# Autodesk Inventor assembly: printer
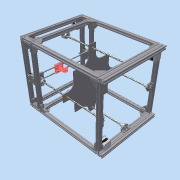
[picture p0: Inventor's stored thumbnail of the model, 180x180]
Saved by Autodesk Inventor 2015 (Build 190159000, 159)
## iProperties
Created: 2016-06-24
Part Number: printer
Document SubType Name: Assembly
Designer: Dustin
Author: Dustin
## Documents named in this file (25)
- E:\Documents\3D Printer\Parts\New Printer\printer.iam
- E:\Documents\3D Printer\Parts\New Printer\20x20x9in.ipt
- E:\Documents\3D Printer\Parts\New Printer\20x20x27cm.ipt
- E:\Documents\3D Printer\Parts\New Printer\heated bed.ipt
- E:\Documents\3D Printer\Parts\New Printer\NEMA17.ipt
- E:\Documents\3D Printer\Parts\New Printer\.375 - 8 (4 start) acme thread.ipt
- E:\Documents\3D Printer\Parts\New Printer\leadscrew corners.ipt
- E:\Documents\3D Printer\Parts\New Printer\bed plate.ipt
- E:\Documents\3D Printer\Parts\New Printer\Imported Components\GT2_20teeth_pulley\GT2_20teeth_pulley.ipt
- E:\Documents\3D Printer\Parts\New Printer\6mm_rod_265.ipt
- E:\Documents\3D Printer\Parts\New Printer\motor mount.ipt
- E:\Documents\3D Printer\Parts\New Printer\20x20x5cm.ipt
- E:\Documents\3D Printer\Parts\New Printer\extruder.iam
- E:\Documents\3D Printer\Parts\New Printer\X smooth mount.ipt
- E:\Documents\3D Printer\Parts\New Printer\m3x20.ipt
- E:\Documents\3D Printer\Parts\New Printer\Corner mount.ipt
- E:\Documents\3D Printer\Parts\New Printer\m4 bearing assembly.iam
- E:\Documents\3D Printer\Parts\New Printer\m4 bearing assembly 30mm.iam
- E:\Documents\3D Printer\Parts\New Printer\KFL08.iam
- E:\Documents\3D Printer\Parts\New Printer\vwheel.iam
- E:\Documents\3D Printer\Parts\New Printer\m5x16m.ipt
- E:\Documents\3D Printer\Parts\New Printer\m8 nut.ipt
- E:\Documents\3D Printer\Parts\New Printer\corners.ipt
- E:\Documents\3D Printer\Parts\New Printer\Corner mount_MIR.ipt
- E:\Documents\3D Printer\Parts\New Printer\corner bracket.ipt
## Components (123 placed, 25 different names)
1. 20x20x9in:2 — Mate:4, Flush:8, Flush:9, Mate:6, Mate:39, Flush:53, Flush:64, Mate:66, Mate:113, Flush:122, Angle:30
2. 20x20x9in:3 — Mate:5, Flush:10, Flush:11, Flush:12, Flush:13, Mate:48, Flush:51, Flush:65, Mate:67, Mate:109, Flush:120
3. 20x20x27cm:3 — Mate:4, Flush:8, Flush:9, Mate:5, Flush:10, Flush:11, Mate:11, Mate:12, Flush:24, Flush:25, Flush:26, Flush:27, Mate:60, Flush:60, Flush:61, Mate:85, Flush:113, Mate:104, Mate:108
4. 20x20x27cm:4 — Mate:6, Flush:12, Flush:13, Mate:10, Mate:13, Flush:21, Flush:22, Flush:23, Flush:28, Flush:29, Mate:54, Flush:54, Flush:62, Mate:61, Flush:63, Mate:68, Mate:111, Flush:121, Flush:123
5. 20x20x27cm:5 — Mate:13, Flush:21, Flush:28, Flush:29, Mate:116, Mate:127
6. 20x20x27cm:6 — Mate:12, Flush:26, Flush:27, Mate:14, Flush:30, Flush:31, Mate:107, Flush:119, Mate:110, Mate:119, Mate:120
7. 20x20x27cm:7 — Mate:11, Flush:24, Flush:25, Mate:122, Flush:127, Mate:125
8. 20x20x27cm:8 — Mate:10, Flush:22, Flush:23, Mate:112, Mate:114, Mate:129, Mate:130, Flush:131
9. 20x20x9in:5 — Mate:40, Flush:47, Flush:48, Flush:73, Flush:105, Mate:117, Flush:124, Mate:118, Flush:125, Mate:142, Flush:136, Mate:144
10. 20x20x9in:6 — Mate:44, Flush:50, Flush:77, Mate:83, Flush:104, Mate:124, Flush:128, Mate:128, Flush:130, Mate:135, Flush:132, Mate:137, Flush:133
11. 20x20x27cm:9 — Mate:14, Flush:30, Flush:31, Mate:42, Flush:49, Mate:74, Mate:75, Flush:74, Flush:75, Flush:76, Angle:29, Mate:121, Flush:126, Mate:123, Mate:139, Flush:134, Mate:149
12. 20x20x27cm:10 — Mate:46, Flush:71, Flush:72, Mate:72, Mate:73, Flush:78, Mate:126, Flush:129, Mate:131, Mate:146, Flush:137, Mate:148, Flush:138
13. heated bed:1 — Mate:58, Tangent:5, Tangent:6, Insert:54, Insert:55, Insert:56, Insert:57
14. NEMA17:1 — Mate:39, Flush:64, Insert:7, Mate:85, Insert:59
15. NEMA17:2 — Flush:65, Insert:6, Insert:20, Insert:21
16. .375 - 8 (4 start) acme thread:1 — Tangent:1, Flush:58, Insert:3, Tangent:18, Tangent:24, Tangent:56, Tangent:64
17. .375 - 8 (4 start) acme thread:2 — Insert:33, Flush:114, Tangent:62, Tangent:63, Tangent:66, Tangent:75
18. .375 - 8 (4 start) acme thread:3 — Tangent:3, Flush:56, Insert:5, Tangent:14, Tangent:58, Tangent:60, Tangent:68
19. .375 - 8 (4 start) acme thread:4 — Tangent:2, Flush:55, Insert:4, Tangent:16, Tangent:21, Tangent:53, Tangent:70
20. leadscrew corners:1 — Mate:40, Flush:47, Tangent:1, Flush:111, Tangent:57
21. leadscrew corners:2 — Mate:42, Flush:48, Flush:110, Tangent:55
22. leadscrew corners:3 — Mate:44, Flush:49, Tangent:3, Flush:112, Tangent:59
23. leadscrew corners:4 — Mate:46, Flush:50, Tangent:2, Flush:109, Tangent:61
24. leadscrew corners:5 — Mate:48, Flush:51, Flush:58, Tangent:18, Mate:67, Flush:115, Tangent:65
25. leadscrew corners:6 — Flush:113, Mate:104, Flush:114, Tangent:62, Flush:116, Tangent:67
26. leadscrew corners:7 — Mate:54, Flush:54, Flush:55, Tangent:16, Mate:68, Flush:118, Tangent:71
27. leadscrew corners:8 — Flush:53, Flush:56, Tangent:14, Mate:66, Flush:117, Tangent:69
28. bed plate:1 — Mate:58, Tangent:5, Tangent:6, Tangent:21, Tangent:24, Tangent:60, Insert:50, Insert:51, Insert:52, Angle:28, Angle:29, Tangent:72, Tangent:73, Tangent:74, Mate:106, Insert:58
29. GT2_20teeth_pulley:1 — Insert:33
30. GT2_20teeth_pulley:2 — Insert:5
31. GT2_20teeth_pulley:3 — Insert:3
32. GT2_20teeth_pulley:4 — Insert:4
33. 20x20x27cm:11 — Mate:60, Flush:60, Flush:61
34. 20x20x27cm:12 — Flush:62, Mate:61, Flush:63
35. GT2_20teeth_pulley:5 — Insert:6
36. GT2_20teeth_pulley:6 — Insert:7
37. 6mm_rod_265:1 — Flush:68, Mate:83, Tangent:22, Tangent:47, Tangent:51, Angle:26, Angle:27
38. 6mm_rod_265:2 — Flush:68, Tangent:23, Tangent:48, Angle:25, Tangent:52
39. NEMA17:3 — Mate:87, Mate:88, Insert:32, Insert:60
40. NEMA17:4 — Insert:23, Insert:24, Mate:90, Tangent:34, Insert:31, Mate:98
41. 20x20x5cm:1 — Flush:71, Flush:72, Mate:72, Mate:143, Mate:147
42. 20x20x5cm:2 — Mate:75, Flush:73, Flush:74, Mate:132, Mate:133, Mate:140, Mate:141, Flush:135
43. 20x20x5cm:3 — Mate:74, Flush:75, Flush:76, Flush:79, Flush:80, Mate:76, Mate:138, Mate:150, Flush:139
44. 20x20x5cm:4 — Mate:73, Flush:77, Flush:78, Mate:77, Flush:81, Flush:82, Mate:136, Mate:145
45. 20x20x27cm:13 — Mate:77, Flush:81, Flush:82, Mate:88, Mate:90
46. 2020x380mm — Flush:79, Flush:80, Mate:76, Mate:78, Flush:83, Flush:84, Mate:79, Flush:85, Flush:86, Flush:92
47. 20x20x9in:7 — Mate:78, Flush:83, Flush:84, Mate:89, Mate:98, Flush:91, Mate:101, Flush:106
48. 20x20x9in:8 — Mate:79, Flush:85, Flush:86, Mate:87, Angle:28, Angle:31, Mate:115, Mate:134
49. motor mount:2 — Insert:20, Insert:21, Flush:123
50. GT2_20teeth_pulley:7 — Insert:32
51. motor mount:3 — Insert:23, Insert:24, Mate:89
52. extruder:1 [sub-assembly] — Tangent:22, Tangent:23, Tangent:35, Angle:11, Tangent:36, Angle:12, Angle:21, Tangent:45, Angle:22, Tangent:46, Flush:100, Flush:101, Flush:106, Flush:107, Angle:27, Flush:108
53. X smooth mount:1 — Angle:13, Tangent:37, Flush:93, Angle:16, Tangent:40, Flush:95, Tangent:51, Angle:25, Flush:104, Tangent:52, Insert:42, Insert:43, Insert:44, Insert:45, Insert:46, Insert:47, Insert:48, Insert:49
54. GT2_20teeth_pulley:8 — Tangent:34, Insert:31
55. m3x20:1 — Tangent:35, Angle:11, Flush:107
56. Corner mount:2 — Flush:91, Mate:101, Flush:92, Angle:14, Tangent:38, Flush:94, Angle:15, Tangent:39, Mate:103
57. m3x20:2 — Tangent:36, Angle:12, Flush:108
58. m4 bearing assembly:1 [sub-assembly] — Angle:13, Tangent:37, Flush:93
59. m4 bearing assembly:2 [sub-assembly] — Angle:14, Tangent:38, Flush:94
60. m4 bearing assembly 30mm:1 [sub-assembly] — Angle:15, Tangent:39, Mate:103
61. m4 bearing assembly 30mm:2 [sub-assembly] — Angle:16, Tangent:40, Flush:95
62. m4 bearing assembly:3 [sub-assembly] — Tangent:50, Angle:24, Flush:103
63. m4 bearing assembly 30mm:3 [sub-assembly] — Tangent:49, Angle:23, Flush:102
64. m4 bearing assembly:4 [sub-assembly]
65. m4 bearing assembly 30mm:4 [sub-assembly]
66. m3x20:3 — Angle:21, Tangent:45, Flush:100
67. m3x20:4 — Angle:22, Tangent:46, Flush:101
68. X smooth mount:2 — Tangent:47, Tangent:48, Tangent:49, Tangent:50, Angle:23, Angle:24, Flush:102, Flush:103, Angle:26, Flush:105, Insert:34, Insert:35, Insert:36, Insert:37, Insert:38, Insert:39, Insert:40, Insert:41
69. KFL08:1 [sub-assembly] — Flush:109, Tangent:53, Tangent:61
70. KFL08:2 [sub-assembly] — Flush:110, Tangent:55, Tangent:63
71. KFL08:3 [sub-assembly] — Flush:111, Tangent:56, Tangent:57
72. KFL08:4 [sub-assembly] — Flush:112, Tangent:58, Tangent:59
73. KFL08:5 [sub-assembly] — Flush:117, Tangent:68, Tangent:69
74. KFL08:6 [sub-assembly] — Flush:118, Tangent:70, Tangent:71
75. KFL08:7 [sub-assembly] — Flush:116, Tangent:66, Tangent:67
76. KFL08:8 [sub-assembly] — Flush:115, Tangent:64, Tangent:65
77. vwheel:1 [sub-assembly] — Insert:37
78. vwheel:2 [sub-assembly] — Insert:34
79. vwheel:3 [sub-assembly] — Insert:36
80. vwheel:4 [sub-assembly] — Insert:35
81. m5x16m:1 — Insert:40
82. m5x16m:2 — Insert:41
83. m5x16m:3 — Insert:39
84. m5x16m:4 — Insert:38
85. vwheel:5 [sub-assembly] — Insert:42
86. vwheel:6 [sub-assembly] — Insert:43
87. vwheel:7 [sub-assembly] — Insert:44
88. vwheel:8 [sub-assembly] — Insert:45
89. m5x16m:5 — Insert:46
90. m5x16m:6 — Insert:47
91. m5x16m:7 — Insert:49
92. m5x16m:8 — Insert:48
93. m8 nut:1 — Insert:50, Tangent:73
94. m8 nut:2 — Insert:51, Tangent:74
95. m8 nut:3 — Insert:52, Tangent:72, Tangent:75
96. m8 nut:4 — Mate:106, Insert:58
97. m3x20:5 — Insert:54
98. m3x20:6 — Insert:57
99. m3x20:7 — Insert:56
100. m3x20:8 — Insert:55
101. corners:1 — Mate:107, Flush:119, Mate:108
102. corners:2 — Mate:109, Mate:110, Flush:120
103. corners:3 — Mate:113, Mate:114, Flush:122
104. corners:4 — Mate:111, Mate:112, Flush:121
105. motor mount:4 — Insert:59, Angle:30
106. motor mount:5 — Insert:60, Angle:31, Mate:115
107. corners:5 — Mate:116, Mate:117, Flush:124
108. corners:6 — Mate:118, Flush:125, Mate:119
109. corners:7 — Mate:126, Flush:129, Mate:127
110. corners:8 — Mate:124, Mate:125, Flush:128
111. corners:9 — Mate:122, Mate:123, Flush:127
112. corners:10 — Mate:120, Mate:121, Flush:126
113. corners:11 — Mate:128, Mate:129, Flush:130
114. corners:12 — Mate:130, Mate:131, Flush:131
115. Corner mount_MIR:1 — Mate:132, Mate:133, Mate:134
116. corner bracket:1 — Mate:135, Flush:132, Mate:136
117. corner bracket:2 — Mate:137, Mate:138, Flush:133
118. corner bracket:3 — Mate:139, Flush:134, Mate:140
119. corner bracket:4 — Mate:141, Mate:142, Flush:135
120. corner bracket:5 — Mate:143, Flush:136, Mate:144
121. corner bracket:6 — Mate:145, Mate:146, Flush:137
122. corner bracket:7 — Mate:147, Mate:148, Flush:138
123. corner bracket:8 — Mate:149, Mate:150, Flush:139
## Relationships (293: Flush 102, Mate 87, Tangent 49, Insert 38, Angle 17)
- Mate:4: 20x20x9in:2 ↔ 20x20x27cm:3
- Flush:8: 20x20x9in:2 ↔ 20x20x27cm:3
- Flush:9: 20x20x9in:2 ↔ 20x20x27cm:3
- Mate:5: 20x20x9in:3 ↔ 20x20x27cm:3
- Flush:10: 20x20x9in:3 ↔ 20x20x27cm:3
- Flush:11: 20x20x9in:3 ↔ 20x20x27cm:3
- Mate:6: 20x20x9in:2 ↔ 20x20x27cm:4
- Flush:12: 20x20x9in:3 ↔ 20x20x27cm:4
- Flush:13: 20x20x9in:3 ↔ 20x20x27cm:4
- [Mate]: 20x20x9in:6 ↔ 20x20x27cm:9
- [Flush]: 20x20x9in:6 ↔ 20x20x27cm:9
- [Flush]: 20x20x9in:6 ↔ 20x20x27cm:9
- [Mate]: 20x20x9in:5 ↔ 20x20x27cm:9
- [Flush]: 20x20x9in:5 ↔ 20x20x27cm:9
- [Flush]: 20x20x9in:5 ↔ 20x20x27cm:9
- [Mate]: 20x20x9in:6 ↔ 20x20x27cm:10
- [Flush]: 20x20x9in:6 ↔ 20x20x27cm:10
- [Flush]: 20x20x9in:6 ↔ 20x20x27cm:10
- [Flush]: 20x20x9in:5 ↔ 20x20x27cm:10
- Mate:10: 20x20x27cm:4 ↔ 20x20x27cm:8
- Mate:11: 20x20x27cm:3 ↔ 20x20x27cm:7
- Mate:12: 20x20x27cm:3 ↔ 20x20x27cm:6
- Mate:13: 20x20x27cm:4 ↔ 20x20x27cm:5
- Flush:21: 20x20x27cm:4 ↔ 20x20x27cm:5
- Flush:22: 20x20x27cm:4 ↔ 20x20x27cm:8
- Flush:23: 20x20x27cm:4 ↔ 20x20x27cm:8
- Flush:24: 20x20x27cm:3 ↔ 20x20x27cm:7
- Flush:25: 20x20x27cm:3 ↔ 20x20x27cm:7
- Flush:26: 20x20x27cm:3 ↔ 20x20x27cm:6
- Flush:27: 20x20x27cm:3 ↔ 20x20x27cm:6
- Flush:28: 20x20x27cm:4 ↔ 20x20x27cm:5
- Flush:29: 20x20x27cm:4 ↔ 20x20x27cm:5
- Mate:14: 20x20x27cm:6 ↔ 20x20x27cm:9
- Flush:30: 20x20x27cm:6 ↔ 20x20x27cm:9
- Flush:31: 20x20x27cm:6 ↔ 20x20x27cm:9
- Mate:39: 20x20x9in:2 ↔ NEMA17:1
- Mate:40: 20x20x9in:5 ↔ leadscrew corners:1
- Flush:47: 20x20x9in:5 ↔ leadscrew corners:1
- Tangent:1: .375 - 8 (4 start) acme thread:1 ↔ leadscrew corners:1
- Mate:42: 20x20x27cm:9 ↔ leadscrew corners:2
- Flush:48: 20x20x9in:5 ↔ leadscrew corners:2
- Mate:44: 20x20x9in:6 ↔ leadscrew corners:3
- Flush:49: 20x20x27cm:9 ↔ leadscrew corners:3
- Mate:46: 20x20x27cm:10 ↔ leadscrew corners:4
- Flush:50: 20x20x9in:6 ↔ leadscrew corners:4
- Tangent:2: .375 - 8 (4 start) acme thread:4 ↔ leadscrew corners:4
- Tangent:3: .375 - 8 (4 start) acme thread:3 ↔ leadscrew corners:3
- Mate:48: 20x20x9in:3 ↔ leadscrew corners:5
- Flush:51: 20x20x9in:3 ↔ leadscrew corners:5
- Flush:53: 20x20x9in:2 ↔ leadscrew corners:8
- Mate:54: 20x20x27cm:4 ↔ leadscrew corners:7
- Flush:54: 20x20x27cm:4 ↔ leadscrew corners:7
- Flush:55 (5 mm): .375 - 8 (4 start) acme thread:4 ↔ leadscrew corners:7
- Flush:56 (5 mm): .375 - 8 (4 start) acme thread:3 ↔ leadscrew corners:8
- Flush:58 (5 mm): .375 - 8 (4 start) acme thread:1 ↔ leadscrew corners:5
- Mate:58 (6 mm): heated bed:1 ↔ bed plate:1
- Tangent:5: heated bed:1 ↔ bed plate:1
- Tangent:6: heated bed:1 ↔ bed plate:1
- Insert:3 (-28 mm): .375 - 8 (4 start) acme thread:1 ↔ GT2_20teeth_pulley:3
- Insert:4 (-28 mm): .375 - 8 (4 start) acme thread:4 ↔ GT2_20teeth_pulley:4
- Insert:5 (-28 mm): .375 - 8 (4 start) acme thread:3 ↔ GT2_20teeth_pulley:2
- Mate:60: 20x20x27cm:3 ↔ 20x20x27cm:11
- Flush:60: 20x20x27cm:3 ↔ 20x20x27cm:11
- Flush:61: 20x20x27cm:3 ↔ 20x20x27cm:11
- Flush:62: 20x20x27cm:4 ↔ 20x20x27cm:12
- Mate:61: 20x20x27cm:4 ↔ 20x20x27cm:12
- Flush:63: 20x20x27cm:4 ↔ 20x20x27cm:12
- Flush:64: 20x20x9in:2 ↔ NEMA17:1
- Flush:65: 20x20x9in:3 ↔ NEMA17:2
- Insert:6 (-14 mm): NEMA17:2 ↔ GT2_20teeth_pulley:5
- Insert:7 (-14 mm): NEMA17:1 ↔ GT2_20teeth_pulley:6
- Flush:68: 6mm_rod_265:1 ↔ 6mm_rod_265:2
- Tangent:14: .375 - 8 (4 start) acme thread:3 ↔ leadscrew corners:8
- Tangent:16 (-1 mm): .375 - 8 (4 start) acme thread:4 ↔ leadscrew corners:7
- Tangent:18: .375 - 8 (4 start) acme thread:1 ↔ leadscrew corners:5
- Mate:66: 20x20x9in:2 ↔ leadscrew corners:8
- Mate:67: 20x20x9in:3 ↔ leadscrew corners:5
- Mate:68: 20x20x27cm:4 ↔ leadscrew corners:7
- Flush:71: 20x20x27cm:10 ↔ 20x20x5cm:1
- Flush:72: 20x20x27cm:10 ↔ 20x20x5cm:1
- Mate:72: 20x20x27cm:10 ↔ 20x20x5cm:1
- Mate:73: 20x20x27cm:10 ↔ 20x20x5cm:4
- Mate:74: 20x20x27cm:9 ↔ 20x20x5cm:3
- Mate:75: 20x20x27cm:9 ↔ 20x20x5cm:2
- Flush:73: 20x20x9in:5 ↔ 20x20x5cm:2
- Flush:74: 20x20x27cm:9 ↔ 20x20x5cm:2
- Flush:75: 20x20x27cm:9 ↔ 20x20x5cm:3
- Flush:76: 20x20x27cm:9 ↔ 20x20x5cm:3
- Flush:77: 20x20x9in:6 ↔ 20x20x5cm:4
- Flush:78: 20x20x27cm:10 ↔ 20x20x5cm:4
- Flush:79: 20x20x5cm:3 ↔ 2020x380mm
- Flush:80: 20x20x5cm:3 ↔ 2020x380mm
- Mate:76: 20x20x5cm:3 ↔ 2020x380mm
- Mate:77: 20x20x5cm:4 ↔ 20x20x27cm:13
- Flush:81: 20x20x5cm:4 ↔ 20x20x27cm:13
- Flush:82: 20x20x5cm:4 ↔ 20x20x27cm:13
- Mate:78: 2020x380mm ↔ 20x20x9in:7
- Flush:83: 2020x380mm ↔ 20x20x9in:7
- Flush:84: 2020x380mm ↔ 20x20x9in:7
- Mate:79: 2020x380mm ↔ 20x20x9in:8
- Flush:85: 2020x380mm ↔ 20x20x9in:8
- Flush:86: 2020x380mm ↔ 20x20x9in:8
- Insert:20: NEMA17:2 ↔ motor mount:2
- Insert:21: NEMA17:2 ↔ motor mount:2
- Tangent:21: .375 - 8 (4 start) acme thread:4 ↔ bed plate:1
- Insert:23: NEMA17:4 ↔ motor mount:3
- Insert:24: NEMA17:4 ↔ motor mount:3
- Mate:83: 20x20x9in:6 ↔ 6mm_rod_265:1
- Tangent:22: 6mm_rod_265:1 ↔ extruder:1
- Tangent:23: 6mm_rod_265:2 ↔ extruder:1
- Mate:85: 20x20x27cm:3 ↔ NEMA17:1
- Tangent:24: .375 - 8 (4 start) acme thread:1 ↔ bed plate:1
- Mate:87: NEMA17:3 ↔ 20x20x9in:8
- Mate:88: NEMA17:3 ↔ 20x20x27cm:13
- Mate:89: 20x20x9in:7 ↔ motor mount:3
- Mate:90: NEMA17:4 ↔ 20x20x27cm:13
- Tangent:34: NEMA17:4 ↔ GT2_20teeth_pulley:8
- Insert:31 (5 mm): NEMA17:4 ↔ GT2_20teeth_pulley:8
- Mate:98: NEMA17:4 ↔ 20x20x9in:7
- Tangent:35: extruder:1 ↔ m3x20:1
- Angle:11 (180 deg): extruder:1 ↔ m3x20:1
- Flush:91: 20x20x9in:7 ↔ Corner mount:2
- Mate:101: 20x20x9in:7 ↔ Corner mount:2
- Flush:92: 2020x380mm ↔ Corner mount:2
- Insert:32: NEMA17:3 ↔ GT2_20teeth_pulley:7
- Tangent:36: extruder:1 ↔ m3x20:2
- Angle:12 (180 deg): extruder:1 ↔ m3x20:2
- Angle:13 (180 deg): X smooth mount:1 ↔ m4 bearing assembly:1
- Tangent:37: X smooth mount:1 ↔ m4 bearing assembly:1
- Flush:93 (-5 mm): X smooth mount:1 ↔ m4 bearing assembly:1
- Angle:14 (0 deg): Corner mount:2 ↔ m4 bearing assembly:2
- Tangent:38: Corner mount:2 ↔ m4 bearing assembly:2
- Flush:94 (-6 mm): Corner mount:2 ↔ m4 bearing assembly:2
- Angle:15 (0 deg): Corner mount:2 ↔ m4 bearing assembly 30mm:1
- Tangent:39: Corner mount:2 ↔ m4 bearing assembly 30mm:1
- Mate:103 (15 mm): Corner mount:2 ↔ m4 bearing assembly 30mm:1
- Angle:16 (180 deg): X smooth mount:1 ↔ m4 bearing assembly 30mm:2
- Tangent:40: X smooth mount:1 ↔ m4 bearing assembly 30mm:2
- Flush:95: X smooth mount:1 ↔ m4 bearing assembly 30mm:2
- Angle:21 (180 deg): extruder:1 ↔ m3x20:3
- Tangent:45: extruder:1 ↔ m3x20:3
- Angle:22 (180 deg): extruder:1 ↔ m3x20:4
- Tangent:46: extruder:1 ↔ m3x20:4
- Flush:100 (-6 mm): extruder:1 ↔ m3x20:3
- Flush:101 (-2 mm): extruder:1 ↔ m3x20:4
- Tangent:47: 6mm_rod_265:1 ↔ X smooth mount:2
- Tangent:48: 6mm_rod_265:2 ↔ X smooth mount:2
- Tangent:49: m4 bearing assembly 30mm:3 ↔ X smooth mount:2
- Tangent:50: m4 bearing assembly:3 ↔ X smooth mount:2
- Angle:23 (180 deg): m4 bearing assembly 30mm:3 ↔ X smooth mount:2
- Angle:24 (180 deg): m4 bearing assembly:3 ↔ X smooth mount:2
- Flush:102 (1 mm): m4 bearing assembly 30mm:3 ↔ X smooth mount:2
- Flush:103 (-5 mm): m4 bearing assembly:3 ↔ X smooth mount:2
- Tangent:51: 6mm_rod_265:1 ↔ X smooth mount:1
- Angle:25 (0 deg): 6mm_rod_265:2 ↔ X smooth mount:1
- Flush:104: 20x20x9in:6 ↔ X smooth mount:1
- Tangent:52: 6mm_rod_265:2 ↔ X smooth mount:1
- Angle:26 (0 deg): 6mm_rod_265:1 ↔ X smooth mount:2
- Flush:105: 20x20x9in:5 ↔ X smooth mount:2
- Flush:106 (47 mm): 20x20x9in:7 ↔ extruder:1
- Flush:107: extruder:1 ↔ m3x20:1
- Angle:27 (0 deg): 6mm_rod_265:1 ↔ extruder:1
- Flush:108 (-5 mm): extruder:1 ↔ m3x20:2
- Flush:109: leadscrew corners:4 ↔ KFL08:1
- Tangent:53: .375 - 8 (4 start) acme thread:4 ↔ KFL08:1
- Flush:110: leadscrew corners:2 ↔ KFL08:2
- Tangent:55: leadscrew corners:2 ↔ KFL08:2
- Flush:111: leadscrew corners:1 ↔ KFL08:3
- Tangent:56: .375 - 8 (4 start) acme thread:1 ↔ KFL08:3
- Tangent:57: leadscrew corners:1 ↔ KFL08:3
- Flush:112: leadscrew corners:3 ↔ KFL08:4
- Tangent:58: .375 - 8 (4 start) acme thread:3 ↔ KFL08:4
- Tangent:59: leadscrew corners:3 ↔ KFL08:4
- Tangent:60 (-1 mm): .375 - 8 (4 start) acme thread:3 ↔ bed plate:1
- Tangent:61: leadscrew corners:4 ↔ KFL08:1
- Flush:113: 20x20x27cm:3 ↔ leadscrew corners:6
- Mate:104: 20x20x27cm:3 ↔ leadscrew corners:6
- Insert:33 (-23 mm): .375 - 8 (4 start) acme thread:2 ↔ GT2_20teeth_pulley:1
- Flush:114 (-5 mm): .375 - 8 (4 start) acme thread:2 ↔ leadscrew corners:6
- Tangent:62: .375 - 8 (4 start) acme thread:2 ↔ leadscrew corners:6
- Tangent:63: .375 - 8 (4 start) acme thread:2 ↔ KFL08:2
- Flush:115: leadscrew corners:5 ↔ KFL08:8
- Tangent:64: .375 - 8 (4 start) acme thread:1 ↔ KFL08:8
- Tangent:65: leadscrew corners:5 ↔ KFL08:8
- Flush:116: leadscrew corners:6 ↔ KFL08:7
- Tangent:66: .375 - 8 (4 start) acme thread:2 ↔ KFL08:7
- Tangent:67: leadscrew corners:6 ↔ KFL08:7
- Flush:117: leadscrew corners:8 ↔ KFL08:5
- Tangent:68: .375 - 8 (4 start) acme thread:3 ↔ KFL08:5
- Tangent:69: leadscrew corners:8 ↔ KFL08:5
- Flush:118: leadscrew corners:7 ↔ KFL08:6
- Tangent:70: .375 - 8 (4 start) acme thread:4 ↔ KFL08:6
- Tangent:71: leadscrew corners:7 ↔ KFL08:6
- Insert:34 (0.4 mm): X smooth mount:2 ↔ vwheel:2
- Insert:35 (0.4 mm): X smooth mount:2 ↔ vwheel:4
- Insert:36 (0.4 mm): X smooth mount:2 ↔ vwheel:3
- Insert:37 (0.4 mm): X smooth mount:2 ↔ vwheel:1
- Insert:38: X smooth mount:2 ↔ m5x16m:4
- Insert:39: X smooth mount:2 ↔ m5x16m:3
- Insert:40: X smooth mount:2 ↔ m5x16m:1
- Insert:41: X smooth mount:2 ↔ m5x16m:2
- Insert:42: X smooth mount:1 ↔ vwheel:5
- Insert:43: X smooth mount:1 ↔ vwheel:6
- Insert:44: X smooth mount:1 ↔ vwheel:7
- Insert:45: X smooth mount:1 ↔ vwheel:8
- Insert:46: X smooth mount:1 ↔ m5x16m:5
- Insert:47: X smooth mount:1 ↔ m5x16m:6
- Insert:48: X smooth mount:1 ↔ m5x16m:8
- Insert:49: X smooth mount:1 ↔ m5x16m:7
- Insert:50: bed plate:1 ↔ m8 nut:1
- Insert:51: bed plate:1 ↔ m8 nut:2
- Insert:52: bed plate:1 ↔ m8 nut:3
- Angle:28 (0 deg): bed plate:1 ↔ 20x20x9in:8
- Angle:29 (0 deg): 20x20x27cm:9 ↔ bed plate:1
- Insert:54: heated bed:1 ↔ m3x20:5
- Insert:55: heated bed:1 ↔ m3x20:8
- Insert:56: heated bed:1 ↔ m3x20:7
- Insert:57: heated bed:1 ↔ m3x20:6
- Tangent:72: bed plate:1 ↔ m8 nut:3
- Tangent:73: bed plate:1 ↔ m8 nut:1
- Tangent:74: bed plate:1 ↔ m8 nut:2
- Mate:106: bed plate:1 ↔ m8 nut:4
- Insert:58: bed plate:1 ↔ m8 nut:4
- Mate:107: 20x20x27cm:6 ↔ corners:1
- Flush:119: 20x20x27cm:6 ↔ corners:1
- Mate:108: 20x20x27cm:3 ↔ corners:1
- Mate:109: 20x20x9in:3 ↔ corners:2
- Mate:110: 20x20x27cm:6 ↔ corners:2
- Flush:120: 20x20x9in:3 ↔ corners:2
- Mate:111: 20x20x27cm:4 ↔ corners:4
- Mate:112: 20x20x27cm:8 ↔ corners:4
- Flush:121: 20x20x27cm:4 ↔ corners:4
- Mate:113: 20x20x9in:2 ↔ corners:3
- Mate:114: 20x20x27cm:8 ↔ corners:3
- Flush:122: 20x20x9in:2 ↔ corners:3
- Flush:123: 20x20x27cm:4 ↔ motor mount:2
- Insert:59: NEMA17:1 ↔ motor mount:4
- Angle:30 (0 deg): 20x20x9in:2 ↔ motor mount:4
- Insert:60: NEMA17:3 ↔ motor mount:5
- Angle:31 (0 deg): 20x20x9in:8 ↔ motor mount:5
- Mate:115: 20x20x9in:8 ↔ motor mount:5
- Mate:116: 20x20x27cm:5 ↔ corners:5
- Mate:117: 20x20x9in:5 ↔ corners:5
- Flush:124: 20x20x9in:5 ↔ corners:5
- Mate:118: 20x20x9in:5 ↔ corners:6
- Flush:125: 20x20x9in:5 ↔ corners:6
- Mate:119: 20x20x27cm:6 ↔ corners:6
- Mate:120: 20x20x27cm:6 ↔ corners:10
- Mate:121: 20x20x27cm:9 ↔ corners:10
- Flush:126: 20x20x27cm:9 ↔ corners:10
- Mate:122: 20x20x27cm:7 ↔ corners:9
- Mate:123: 20x20x27cm:9 ↔ corners:9
- Flush:127: 20x20x27cm:7 ↔ corners:9
- Mate:124: 20x20x9in:6 ↔ corners:8
- Mate:125: 20x20x27cm:7 ↔ corners:8
- Flush:128: 20x20x9in:6 ↔ corners:8
- Mate:126: 20x20x27cm:10 ↔ corners:7
- Flush:129: 20x20x27cm:10 ↔ corners:7
- Mate:127: 20x20x27cm:5 ↔ corners:7
- Mate:128: 20x20x9in:6 ↔ corners:11
- Mate:129: 20x20x27cm:8 ↔ corners:11
- Flush:130: 20x20x9in:6 ↔ corners:11
- Mate:130: 20x20x27cm:8 ↔ corners:12
- Mate:131: 20x20x27cm:10 ↔ corners:12
- Flush:131: 20x20x27cm:8 ↔ corners:12
- Mate:132: 20x20x5cm:2 ↔ Corner mount_MIR:1
- Mate:133: 20x20x5cm:2 ↔ Corner mount_MIR:1
- Mate:134: 20x20x9in:8 ↔ Corner mount_MIR:1
- Mate:135: 20x20x9in:6 ↔ corner bracket:1
- Flush:132: 20x20x9in:6 ↔ corner bracket:1
- Mate:136: 20x20x5cm:4 ↔ corner bracket:1
- Mate:137: 20x20x9in:6 ↔ corner bracket:2
- Mate:138: 20x20x5cm:3 ↔ corner bracket:2
- Flush:133: 20x20x9in:6 ↔ corner bracket:2
- Mate:139: 20x20x27cm:9 ↔ corner bracket:3
- Flush:134: 20x20x27cm:9 ↔ corner bracket:3
- Mate:140: 20x20x5cm:2 ↔ corner bracket:3
- Mate:141: 20x20x5cm:2 ↔ corner bracket:4
- Mate:142: 20x20x9in:5 ↔ corner bracket:4
- Flush:135: 20x20x5cm:2 ↔ corner bracket:4
- Mate:143: 20x20x5cm:1 ↔ corner bracket:5
- Flush:136: 20x20x9in:5 ↔ corner bracket:5
- Mate:144: 20x20x9in:5 ↔ corner bracket:5
- Mate:145: 20x20x5cm:4 ↔ corner bracket:6
- Mate:146: 20x20x27cm:10 ↔ corner bracket:6
- Flush:137: 20x20x27cm:10 ↔ corner bracket:6
- Mate:147: 20x20x5cm:1 ↔ corner bracket:7
- Mate:148: 20x20x27cm:10 ↔ corner bracket:7
- Flush:138: 20x20x27cm:10 ↔ corner bracket:7
- Mate:149: 20x20x27cm:9 ↔ corner bracket:8
- Mate:150: 20x20x5cm:3 ↔ corner bracket:8
- Flush:139: 20x20x5cm:3 ↔ corner bracket:8
- Tangent:75: .375 - 8 (4 start) acme thread:2 ↔ m8 nut:3
## Named parameters: d25_d15 = 0 mm, d26_d6 = 0 mm, d27_d7 = 0 mm, d28_d8 = 0 mm, d29_d9 = 0 mm, d30_d10 = 0 mm, d31_d11 = 0 mm, d32_d12 = 0 mm, d33_d13 = 0 mm, d34_d14 = 0 mm
